# Autodesk Inventor assembly: EL2-.200
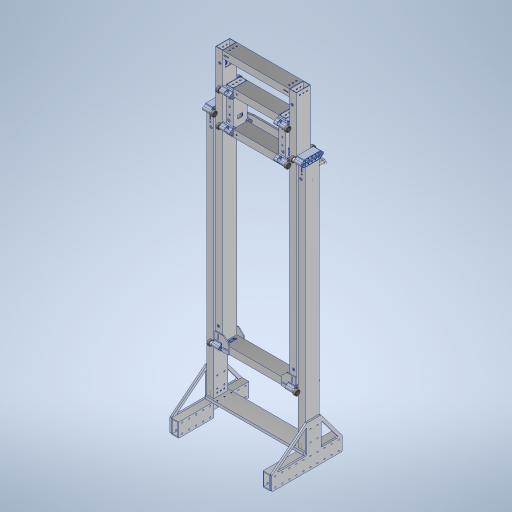
[picture p0: Inventor's stored thumbnail of the model, 512x512]
Saved by Autodesk Inventor 2023.4 (Build 274418000, 418)
## iProperties
Created: 2025-01-11
Part Number: EL2-.200
Document SubType Name: Assembly
Designer: slick
Author: slick
## Documents named in this file (10)
- C:\Users\mavericks\Desktop\2025-ReefScape---CAD\Elevator\EL2\EL2-.200.iam
- C:\Users\mavericks\Desktop\2025-ReefScape---CAD\Elevator\EL2\EL2-003.ipt
- C:\Users\mavericks\Desktop\2025-ReefScape---CAD\Elevator\EL2\EL2-.100.iam
- C:\Users\mavericks\Desktop\2025-ReefScape---CAD\Elevator\EL2\EL2-.300.iam
- C:\Users\mavericks\Desktop\2025-ReefScape---CAD\Elevator\EL2\EL2-C-100.iam
- C:\Users\mavericks\Desktop\2025-ReefScape---CAD\Elevator\EL2\EL2-012.ipt
- C:\Users\mavericks\Desktop\2025-ReefScape---CAD\Elevator\EL2\EL2-013.ipt
- C:\Users\mavericks\Desktop\2025-ReefScape---CAD\Elevator\EL2\EL2-S-002.ipt
- C:\Users\mavericks\Desktop\2025-ReefScape---CAD\Elevator\EL2\EL2-S-001.ipt
- C:\Users\mavericks\Desktop\2025-ReefScape---CAD\Elevator\EL2\EL2-S-003.ipt
## Components (14 placed, 9 different names)
1. EL2-003:1 — Insert:1, Insert:2, Insert:3, Insert:4, Mate:3
2. EL2-.100:1 [sub-assembly] — Insert:1, Insert:3, Symmetry:1, Mate:2, Insert:10, Insert:19, Insert:22
3. EL2-.100:2 [sub-assembly] — Insert:2, Insert:4, Symmetry:1, Insert:9, Insert:20, Insert:21
4. EL2-.300:1 [sub-assembly] — Mate:1, Mate:2, Mate:3, Mate:4, Mate:5, Mate:6
5. EL2-C-100:1 [sub-assembly] — Mate:4, Mate:5, Mate:6
6. EL2-012:1 — Insert:7, Insert:9
7. EL2-012:2 — Insert:8, Insert:10
8. EL2-013:1 — Insert:7, Insert:8
9. EL2-S-002:1 — Insert:15, Insert:20, Insert:21, Insert:25, Insert:26, Insert:27
10. EL2-S-002:2 — Insert:19, Insert:22, Insert:23, Insert:24, Insert:28, Insert:29
11. EL2-S-001:1 — Insert:23, Insert:24
12. EL2-S-001:2 — Insert:15, Insert:25
13. EL2-S-003:1 — Insert:26, Insert:27
14. EL2-S-003:2 — Insert:28, Insert:29
## Relationships (27: Insert 20, Mate 6, Symmetry 1)
- Insert:1: EL2-003:1 ↔ EL2-.100:1
- Insert:2: EL2-003:1 ↔ EL2-.100:2
- Insert:3: EL2-003:1 ↔ EL2-.100:1
- Insert:4: EL2-003:1 ↔ EL2-.100:2
- Symmetry:1: EL2-.100:1 ↔ EL2-.100:2
- Mate:1: EL2-.300:1
- Mate:2: EL2-.100:1 ↔ EL2-.300:1
- Mate:3: EL2-003:1 ↔ EL2-.300:1
- Mate:4: EL2-.300:1 ↔ EL2-C-100:1
- Mate:5: EL2-.300:1 ↔ EL2-C-100:1
- Mate:6: EL2-.300:1 ↔ EL2-C-100:1
- Insert:7: EL2-012:1 ↔ EL2-013:1
- Insert:8: EL2-012:2 ↔ EL2-013:1
- Insert:9: EL2-.100:2 ↔ EL2-012:1
- Insert:10: EL2-.100:1 ↔ EL2-012:2
- Insert:15: EL2-S-002:1 ↔ EL2-S-001:2
- Insert:19: EL2-.100:1 ↔ EL2-S-002:2
- Insert:20: EL2-.100:2 ↔ EL2-S-002:1
- Insert:21: EL2-.100:2 ↔ EL2-S-002:1
- Insert:22: EL2-.100:1 ↔ EL2-S-002:2
- Insert:23: EL2-S-002:2 ↔ EL2-S-001:1
- Insert:24: EL2-S-002:2 ↔ EL2-S-001:1
- Insert:25: EL2-S-002:1 ↔ EL2-S-001:2
- Insert:26: EL2-S-002:1 ↔ EL2-S-003:1
- Insert:27: EL2-S-002:1 ↔ EL2-S-003:1
- Insert:28: EL2-S-002:2 ↔ EL2-S-003:2
- Insert:29: EL2-S-002:2 ↔ EL2-S-003:2
